# Autodesk Inventor assembly: manipulator
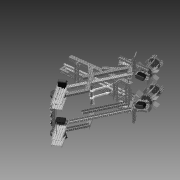
[picture p0: Inventor's stored thumbnail of the model, 180x180]
Saved by Autodesk Inventor 2014 SP1 (Build 180222100, 222)
## iProperties
Created: 2014-03-11
Part Number: manipulator
Document SubType Name: Assembly
Designer: Ryan
Author: Ryan
## Documents named in this file (7)
- C:\Users\Ryan\Desktop\sw\toss up 4th robot\manipulator\manipulator.iam
- C:\Users\Ryan\Desktop\sw\toss up 4th robot\intake\intake.iam
- C:\Users\Ryan\Desktop\sw\toss up 4th robot\6 bar\6 bar.iam
- C:\Users\Ryan\Desktop\sw\toss up 4th robot\6 bar\6 bar_MIR.iam
- C:\Users\Ryan\Desktop\sw\toss up 4th robot\tower\one side of tower.iam
- C:\Users\Ryan\Desktop\sw\toss up 4th robot\tower\one side of tower_MIR.iam
- C:\Users\Ryan\Desktop\sw\toss up 4th robot\buttons.iam
## Components (6 placed, 6 different names)
1. intake:1 [sub-assembly] — Mate:3, Mate:4, Mate:5, Mate:6, Mate:7, Mate:8
2. 6 bar:1 [sub-assembly] — Mate:3, Mate:4, Mate:5, Mate:9, Mate:10, Mate:11
3. 6 bar_MIR:1 [sub-assembly] — Mate:6, Mate:7, Mate:8, Mate:12, Mate:13, Mate:14
4. one side of tower:1 [sub-assembly] — Mate:9, Mate:10, Mate:11, Flush:1
5. one side of tower_MIR:1 [sub-assembly] — Mate:12, Mate:13, Mate:14, Flush:1, Mate:15, Flush:2, Flush:3
6. buttons:1 [sub-assembly] — Mate:15, Flush:2, Flush:3
## Relationships (16: Mate 13, Flush 3)
- Mate:3 (4.7625 mm): intake:1 ↔ 6 bar:1
- Mate:4: intake:1 ↔ 6 bar:1
- Mate:5: intake:1 ↔ 6 bar:1
- Mate:6 (4.7625 mm): intake:1 ↔ 6 bar_MIR:1
- Mate:7: intake:1 ↔ 6 bar_MIR:1
- Mate:8: intake:1 ↔ 6 bar_MIR:1
- Mate:9: 6 bar:1 ↔ one side of tower:1
- Mate:10: 6 bar:1 ↔ one side of tower:1
- Mate:11: 6 bar:1 ↔ one side of tower:1
- Mate:12: 6 bar_MIR:1 ↔ one side of tower_MIR:1
- Mate:13: 6 bar_MIR:1 ↔ one side of tower_MIR:1
- Mate:14: 6 bar_MIR:1 ↔ one side of tower_MIR:1
- Flush:1: one side of tower:1 ↔ one side of tower_MIR:1
- Mate:15: one side of tower_MIR:1 ↔ buttons:1
- Flush:2: one side of tower_MIR:1 ↔ buttons:1
- Flush:3: one side of tower_MIR:1 ↔ buttons:1
